# Autodesk Inventor assembly: Mouse
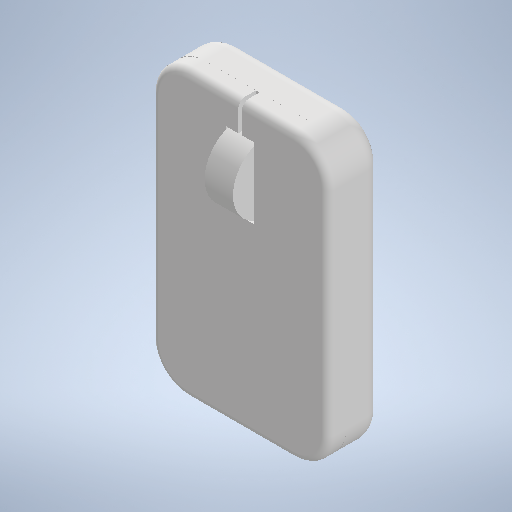
[picture p0: Inventor's stored thumbnail of the model, 512x512]
Saved by Autodesk Inventor 2025 (Build 290162010, 162A)
## iProperties
Created: 2025-10-21
Part Number: Mouse
Document SubType Name: Assembly
Designer: 202321250026
Author: 202321250026
## Documents named in this file (4)
- D:\Users\202321250026\Documents\Github\eng-comp\desenho-assistido\Inventor\Aula_02\Mouse.iam
- D:\Users\202321250026\Documents\Github\eng-comp\desenho-assistido\Inventor\Aula_02\Carcaca-Baixa.ipt
- D:\Users\202321250026\Documents\Github\eng-comp\desenho-assistido\Inventor\Aula_02\Placa-Circuito.ipt
- D:\Users\202321250026\Documents\Github\eng-comp\desenho-assistido\Inventor\Aula_02\Tampa.ipt
## Components (3 placed, 3 different names)
1. Carcaca-Baixa:1 — Alinhado:1, Alinhado:2
2. Placa-Circuito:1 — Alinhado:1
3. Tampa:1 — Alinhado:2
## Relationships (2: Flush 2)
- Alinhado:1 [Flush]: Carcaca-Baixa:1 ↔ Placa-Circuito:1
- Alinhado:2 [Flush]: Carcaca-Baixa:1 ↔ Tampa:1
